# Autodesk Inventor assembly: Montagem1
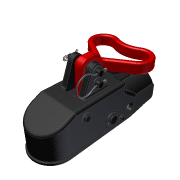
[picture p0: Inventor's stored thumbnail of the model, 180x180]
Saved by Autodesk Inventor 2012 SP2 (Build 160219200, 219)
## iProperties
Created: 2015-05-25
Part Number: Montagem1
Document SubType Name: Assembly
Designer: Projeto02
Author: Projeto02
## Documents named in this file (15)
- C:\Users\Projeto02\Desktop\munheca_engate\Montagem1.iam
- C:\Users\Projeto02\Desktop\munheca_engate\parte_3.ipt
- C:\Users\Projeto02\Desktop\munheca_engate\parte_2.ipt
- C:\Users\Projeto02\Desktop\munheca_engate\pino_a2.ipt
- C:\Users\Projeto02\Desktop\munheca_engate\pino_a3.ipt
- C:\Users\Projeto02\Desktop\munheca_engate\parte_1.ipt
- C:\Users\Projeto02\Desktop\munheca_engate\parte_4.ipt
- C:\Users\Projeto02\Desktop\munheca_engate\pino_b2.ipt
- C:\Users\Projeto02\Desktop\munheca_engate\pino_b1.ipt
- C:\Users\Projeto02\Desktop\munheca_engate\pino_a1.ipt
- C:\Users\Projeto02\Desktop\munheca_engate\anel_1.ipt
- C:\Users\Projeto02\Desktop\munheca_engate\anel_2.ipt
- C:\Users\Projeto02\Desktop\munheca_engate\anel_3.ipt
- C:\Users\Projeto02\Desktop\munheca_engate\contra_pino_1.ipt
- C:\Users\Projeto02\Desktop\munheca_engate\cabo_aco_1.ipt
## Components (20 placed, 14 different names)
1. parte_1:1 — Coincidência:3, Coincidência:4, Coincidência:5, Coincidência:7, Coincidência:8, Coincidência:10, Ângulo:2, Ângulo:3, Ângulo:5, Ângulo:6, Coincidência:6, Alinhamento:6, Alinhamento:7, Alinhamento:11, Alinhamento:12, Alinhamento:13, Alinhamento:14
2. parte_2:1 — Coincidência:1, Ângulo:4, Alinhamento:5
3. parte_3:1 — Coincidência:2, Ângulo:3, Ângulo:4, Alinhamento:3
4. pino_a1:1 — Coincidência:10, Coincidência:18, Coincidência:20, Coincidência:19, Coincidência:21, Alinhamento:11
5. pino_a2:1 — Coincidência:2, Coincidência:3, Coincidência:12, Ângulo:2, Coincidência:13, Coincidência:25, Coincidência:24, Alinhamento:3, Alinhamento:7
6. pino_a3:1 — Coincidência:1, Coincidência:4, Coincidência:11, Coincidência:27, Coincidência:26, Alinhamento:5, Alinhamento:6
7. parte_4:1 — Coincidência:5, Coincidência:9, Coincidência:6
8. pino_b1:1 — Coincidência:7, Coincidência:9, Coincidência:15, Coincidência:28, Coincidência:30, Tangente:1, Coincidência:16, Alinhamento:13
9. pino_b2:1 — Coincidência:8, Coincidência:14, Coincidência:29, Coincidência:23, Coincidência:17, Coincidência:22, Alinhamento:12
10. contra_pino_1:1 — Coincidência:28, Ângulo:6, Tangente:1
11. cabo_aco_1:1 — Coincidência:29, Coincidência:30, Ângulo:5, Alinhamento:14
12. anel_1:1 — Coincidência:11
13. anel_2:3 — Coincidência:12, Coincidência:13
14. anel_2:1 — Coincidência:14, Coincidência:17
15. anel_2:2 — Coincidência:15, Coincidência:16
16. anel_3:1 — Coincidência:18, Coincidência:19
17. anel_3:2 — Coincidência:20, Coincidência:21
18. anel_2:4 — Coincidência:23, Coincidência:22
19. anel_2:5 — Coincidência:25, Coincidência:24
20. anel_1:2 — Coincidência:27, Coincidência:26
## Relationships (44: Mate 30, Flush 8, Angle 5, Tangent 1)
- Coincidência:1 [Mate]: parte_2:1 ↔ pino_a3:1
- Ângulo:4 [Angle] (0 deg): parte_2:1 ↔ parte_3:1
- Coincidência:2 [Mate]: parte_3:1 ↔ pino_a2:1
- Coincidência:3 [Mate]: parte_1:1 ↔ pino_a2:1
- Coincidência:7 [Mate]: parte_1:1 ↔ pino_b1:1
- Coincidência:8 [Mate]: parte_1:1 ↔ pino_b2:1
- Coincidência:14 [Mate]: pino_b2:1 ↔ anel_2:1
- Coincidência:10 [Mate]: parte_1:1 ↔ pino_a1:1
- Coincidência:12 [Mate]: pino_a2:1 ↔ anel_2:3
- Ângulo:2 [Angle] (0 deg): parte_1:1 ↔ pino_a2:1
- Coincidência:4 [Mate]: parte_1:1 ↔ pino_a3:1
- Coincidência:11 [Mate]: pino_a3:1 ↔ anel_1:1
- Coincidência:5 [Mate]: parte_1:1 ↔ parte_4:1
- Coincidência:27 [Mate]: pino_a3:1 ↔ anel_1:2
- Coincidência:26 [Mate]: pino_a3:1 ↔ anel_1:2
- Alinhamento:5 [Flush] (15 mm): parte_2:1 ↔ pino_a3:1
- Ângulo:3 [Angle] (0 deg): parte_1:1 ↔ parte_3:1
- Ângulo:5 [Angle] (0 deg): parte_1:1 ↔ cabo_aco_1:1
- Ângulo:6 [Angle] (0 deg): parte_1:1 ↔ contra_pino_1:1
- Coincidência:6 [Mate] (4.75 mm): parte_1:1 ↔ parte_4:1
- Alinhamento:6 [Flush] (4.25 mm): parte_1:1 ↔ pino_a3:1
- Alinhamento:7 [Flush] (4.5 mm): parte_1:1 ↔ pino_a2:1
- Coincidência:13 [Mate]: pino_a2:1 ↔ anel_2:3
- Coincidência:25 [Mate]: pino_a2:1 ↔ anel_2:5
- Coincidência:24 [Mate]: pino_a2:1 ↔ anel_2:5
- Alinhamento:3 [Flush] (14.375 mm): parte_3:1 ↔ pino_a2:1
- Coincidência:9 [Mate]: parte_4:1 ↔ pino_b1:1
- Coincidência:15 [Mate]: pino_b1:1 ↔ anel_2:2
- Coincidência:28 [Mate]: pino_b1:1 ↔ contra_pino_1:1
- Coincidência:30 [Mate]: pino_b1:1 ↔ cabo_aco_1:1
- Tangente:1 (7 mm): pino_b1:1 ↔ contra_pino_1:1
- Coincidência:16 [Mate]: pino_b1:1 ↔ anel_2:2
- Coincidência:29 [Mate]: pino_b2:1 ↔ cabo_aco_1:1
- Coincidência:23 [Mate]: pino_b2:1 ↔ anel_2:4
- Coincidência:17 [Mate]: pino_b2:1 ↔ anel_2:1
- Coincidência:18 [Mate]: pino_a1:1 ↔ anel_3:1
- Coincidência:20 [Mate]: pino_a1:1 ↔ anel_3:2
- Coincidência:19 [Mate]: pino_a1:1 ↔ anel_3:1
- Coincidência:21 [Mate]: pino_a1:1 ↔ anel_3:2
- Alinhamento:11 [Flush] (4.5 mm): parte_1:1 ↔ pino_a1:1
- Coincidência:22 [Mate]: pino_b2:1 ↔ anel_2:4
- Alinhamento:12 [Flush] (7.25 mm): parte_1:1 ↔ pino_b2:1
- Alinhamento:13 [Flush] (7.25 mm): parte_1:1 ↔ pino_b1:1
- Alinhamento:14 [Flush] (33.5 mm): parte_1:1 ↔ cabo_aco_1:1
